# Autodesk Inventor assembly: Assemblyv2
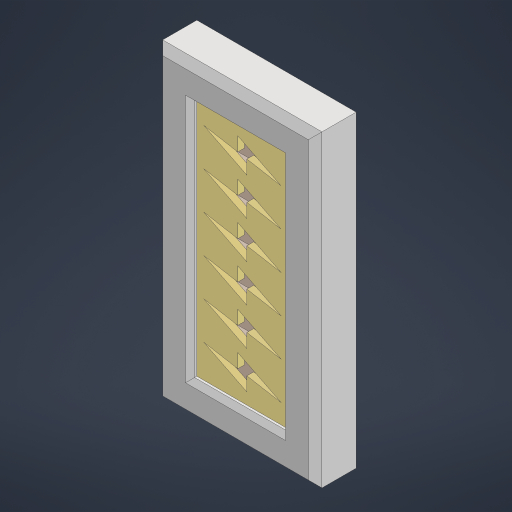
[picture p0: Inventor's stored thumbnail of the model, 512x512]
Saved by Autodesk Inventor 2024.3 (Build 283343000, 343)
## iProperties
Created: 2025-08-11
Part Number: Assemblyv2
Document SubType Name: Assembly
Designer: giuseppe
Author: giuseppe
## Documents named in this file (4)
- C:\Users\giuseppe\Desktop\Buckshot-Ruolette\CAD\counter\V2\Assemblyv2.iam
- C:\Users\giuseppe\Desktop\Buckshot-Ruolette\CAD\counter\panel.ipt
- C:\Users\giuseppe\Desktop\Buckshot-Ruolette\CAD\counter\V2\base.ipt
- C:\Users\giuseppe\Desktop\Buckshot-Ruolette\CAD\counter\V2\fixture.ipt
## Components (3 placed, 3 different names)
1. panel:1 — Flush:1, Flush:2, Flush:3, Flush:4
2. base:1 — Flush:1, Flush:2
3. fixture:1 — Flush:3, Flush:4
## Relationships (4: Flush 4)
- Flush:1: panel:1 ↔ base:1
- Flush:2: panel:1 ↔ base:1
- Flush:3: panel:1 ↔ fixture:1
- Flush:4 (5 mm): panel:1 ↔ fixture:1
